# Autodesk Inventor assembly: Top Crossbrace
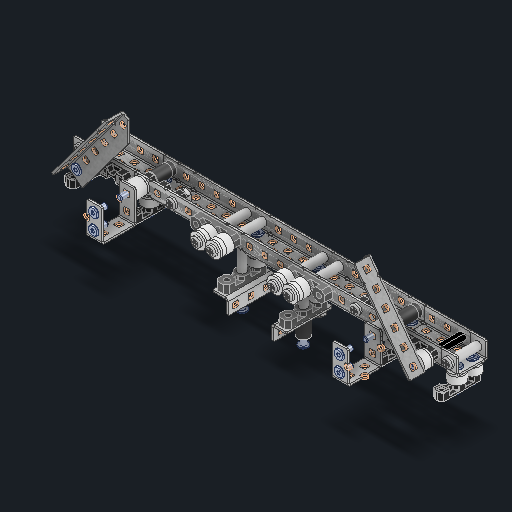
[picture p0: Inventor's stored thumbnail of the model, 512x512]
Saved by Autodesk Inventor 2025.1 (Build 291241000, 241)
## iProperties
Created: 2024-10-20
Part Number: Top Crossbrace
Document SubType Name: Assembly
Designer: Averey Ku
Author: Averey Ku
## Documents named in this file (41)
- C:\Users\avere\VEX\High Stakes\CAD\V3\Chassis\Structure\Top Crossbrace.iam
- C:\Users\avere\VEX\High Stakes\CAD\ROBOPROS-CAD-Inventor\Structure\C Channel\Aluminum 1x2x1\Alu C 1x2x1x17.ipt
- C:\Users\avere\VEX\High Stakes\CAD\ROBOPROS-CAD-Inventor\Structure\C Channel\Aluminum 2x2x2\Alu C 2x2x2x1.ipt
- C:\Users\avere\VEX\High Stakes\CAD\ROBOPROS-CAD-Inventor\Motion\Spacers\Spacer Nylon .500 OD\NSpacer White .500 OD x .375.ipt
- C:\Users\avere\VEX\High Stakes\CAD\ROBOPROS-CAD-Inventor\Motion\Shaft LS\Bearing Flat Low Profile.ipt
- C:\Users\avere\VEX\High Stakes\CAD\ROBOPROS-CAD-Inventor\Motion\Spacers\Washer Steel\SWasher .500 OD x .062500\SWasher .500 OD x .062500.ipt
- C:\Users\avere\VEX\High Stakes\CAD\ROBOPROS-CAD-Inventor\Motion\Spacers\Spacer Nylon .375 OD\NSpacer .375 OD x .125.ipt
- C:\Users\avere\VEX\High Stakes\CAD\ROBOPROS-CAD-Inventor\Motion\Spacers\Spacer Nylon .375 OD\NSpacer .375 OD x .500.ipt
- C:\Users\avere\VEX\High Stakes\CAD\ROBOPROS-CAD-Inventor\Structure\Hardware\Screw Steel - Star\SScrew Star Smooth 1.750.ipt
- C:\Users\avere\VEX\High Stakes\CAD\ROBOPROS-CAD-Inventor\Structure\Hardware\Screw Shoulder Robosource\SScrew Shoulder Smooth .375 x .12.ipt
- C:\Users\avere\VEX\High Stakes\CAD\ROBOPROS-CAD-Inventor\Motion\Spacers\Spacer Nylon .500 OD\NSpacer White .500 OD x .250.ipt
- C:\Users\avere\VEX\High Stakes\CAD\ROBOPROS-CAD-Inventor\Structure\Hardware\Screw Steel - Star\SScrew Star Smooth .750.ipt
- C:\Users\avere\VEX\High Stakes\CAD\ROBOPROS-CAD-Inventor\Structure\C Channel\Aluminum 1x2x1\Alu C 1x2x1x23.ipt
- C:\Users\avere\VEX\High Stakes\CAD\ROBOPROS-CAD-Inventor\Structure\Standoff\Standoff .875.ipt
- C:\Users\avere\VEX\High Stakes\CAD\ROBOPROS-CAD-Inventor\Structure\C Channel\Aluminum 1x3x1 Half Thick Cut\Alu C Half Thick 1x3x1x6.ipt
- C:\Users\avere\VEX\High Stakes\CAD\ROBOPROS-CAD-Inventor\Structure\Hardware\Screw Steel - Star\SScrew Star Smooth .875.ipt
- C:\Users\avere\VEX\High Stakes\CAD\ROBOPROS-CAD-Inventor\Structure\Hardware\Screw Steel - Star\SScrew Star Smooth .290.ipt
- C:\Users\avere\VEX\High Stakes\CAD\V3\Chassis\Structure\Right\Alu C 2x2x2x1 Right.ipt
- C:\Users\avere\VEX\High Stakes\CAD\V3\Chassis\Structure\Right\Bearing Flat Low Profile Right.ipt
- C:\Users\avere\VEX\High Stakes\CAD\V3\Chassis\Structure\Right\Alu C Half Thick 1x3x1x6 Right.ipt
- C:\Users\avere\VEX\High Stakes\CAD\ROBOPROS-CAD-Inventor\Motion\Spacers\Spacer Nylon .500 OD.ipt
- C:\Users\avere\VEX\High Stakes\CAD\ROBOPROS-CAD-Inventor\Motion\Spacers\Washer Steel\SWasher .500 OD x .062500.ipt
- C:\Users\avere\VEX\High Stakes\CAD\ROBOPROS-CAD-Inventor\Motion\Spacers\Spacer Nylon .375 OD.ipt
- C:\Users\avere\VEX\High Stakes\CAD\ROBOPROS-CAD-Inventor\Structure\Hardware\Screw Steel - Star.ipt
- C:\Users\avere\VEX\High Stakes\CAD\ROBOPROS-CAD-Inventor\Structure\Hardware\Screw Shoulder Robosource.ipt
- C:\Users\avere\VEX\High Stakes\CAD\ROBOPROS-CAD-Inventor\Structure\Standoff.ipt
- C:\Users\avere\VEX\High Stakes\CAD\ROBOPROS-CAD-Inventor\Motion\Spacers\Spacer Nylon .500 OD\NSpacer White .500 OD x .500.ipt
- C:\Users\avere\VEX\High Stakes\CAD\ROBOPROS-CAD-Inventor\Structure\Angle\Aluminum 1x1\Alu Angle 1x1x3.ipt
- C:\Users\avere\VEX\High Stakes\CAD\ROBOPROS-CAD-Inventor\Motion\Shaft LS\Bearing Flat.ipt
- C:\Users\avere\VEX\High Stakes\CAD\ROBOPROS-CAD-Inventor\Structure\C Channel\Aluminum 1x2x1\Alu C 1x2x1x25.ipt
- C:\Users\avere\VEX\High Stakes\CAD\ROBOPROS-CAD-Inventor\Structure\Nylon Standoff Rounded\Nylon Standoff .750.ipt
- C:\Users\avere\VEX\High Stakes\CAD\ROBOPROS-CAD-Inventor\Structure\Hardware\Screw Steel - Star\SScrew Star Smooth .250.ipt
- C:\Users\avere\VEX\High Stakes\CAD\ROBOPROS-CAD-Inventor\Structure\Hardware\Screw Steel - Star\SScrew Star Smooth 1.250.ipt
- C:\Users\avere\VEX\High Stakes\CAD\ROBOPROS-CAD-Inventor\Structure\Hardware\Nut Nylon Thread-Forming.ipt
- C:\Users\avere\VEX\High Stakes\CAD\ROBOPROS-CAD-Inventor\Structure\Hardware\Screw Steel - Star\SScrew Star Smooth 1.500.ipt
- C:\Users\avere\VEX\High Stakes\CAD\ROBOPROS-CAD-Inventor\Structure\Nylon Standoff Rounded\Nylon Standoff .875.ipt
- C:\Users\avere\VEX\High Stakes\CAD\ROBOPROS-CAD-Inventor\Structure\Hardware\Screw Nylon - Pan Head\NScrew Pan Head Threaded .250.ipt
- C:\Users\avere\VEX\High Stakes\CAD\ROBOPROS-CAD-Inventor\Structure\Hardware\Screw Nylon - Pan Head\NScrew Pan Head Threaded 1.000.ipt
- C:\Users\avere\VEX\High Stakes\CAD\ROBOPROS-CAD-Inventor\Structure\Hardware\Screw Nylon - Pan Head\NScrew Pan Head Threaded .500.ipt
- C:\Users\avere\VEX\High Stakes\CAD\ROBOPROS-CAD-Inventor\Structure\Hardware\Nut Nylon\Nut Nylon - White.ipt
- C:\Users\avere\VEX\High Stakes\CAD\ROBOPROS-CAD-Inventor\Structure\Hardware\Nut Nylon.ipt
## Components (119 placed, 33 different names)
1. Alu C 1x2x1x23:1 — Insert:23, Flush:2, Insert:33, Insert:34, Mate:6, Insert:39, Insert:40, Insert:79, Mate:12, Insert:80, Mate:13, Mate:14
2. Alu C 1x2x1x17:1 — Insert:3, Insert:5, Mate:2, Insert:15, Flush:1, Flush:2
3. NSpacer White .500 OD x .500:24 — Mate:10, Insert:116, Insert:123
4. Alu Angle 1x1x3:1 — Mate:9, Insert:115, Mate:16, Insert:119, Insert:129
5. NSpacer White .500 OD x .500:28 — Mate:9, Insert:114, Insert:124
6. Alu Angle 1x1x3:2 — Mate:10, Insert:118, Mate:17, Insert:120, Insert:130
7. Bearing Flat:1 — Insert:77, Insert:78, Insert:80, Mate:13
8. Bearing Flat:2 — Insert:75, Insert:76, Insert:79
9. NSpacer White .500 OD x .250:29 — Insert:76, Insert:88
10. NSpacer White .500 OD x .250:30 — Insert:75, Mate:12, Insert:85
11. NSpacer White .500 OD x .250:31 — Insert:78, Insert:92
12. NSpacer White .500 OD x .250:32 — Insert:77, Insert:90
13. NSpacer White .500 OD x .375:33 — Insert:85, Insert:86
14. SWasher .500 OD x .062500:6 — Insert:86, Insert:150
15. NSpacer White .500 OD x .375:35 — Insert:88
16. SWasher .500 OD x .062500:7 — Insert:149
17. NSpacer White .500 OD x .375:36 — Insert:90
18. SWasher .500 OD x .062500:8 — Insert:148
19. NSpacer White .500 OD x .375:37 — Insert:92
20. SWasher .500 OD x .062500:9 — Insert:147
21. Alu C 1x2x1x25:1 — Insert:97, Mate:14, Insert:98, Insert:99, Insert:100, Insert:101, Insert:102, Insert:103, Insert:104, Mate:15, Insert:114, Insert:116, Insert:121, Insert:122, Insert:125, Insert:126, Insert:127, Insert:128, Insert:133, Insert:134, Insert:135, Insert:136, Insert:137, Insert:138, Insert:139, Insert:140, Insert:141, Insert:142, Insert:143, Insert:144, Insert:145, Insert:146, Insert:152, Insert:153
22. SWasher .500 OD x .062500:10 — Insert:106
23. SWasher .500 OD x .062500:11 — Insert:105
24. SWasher .500 OD x .062500:12 — Insert:107
25. SWasher .500 OD x .062500:13 — Insert:108
26. SWasher .500 OD x .062500:14 — Insert:110
27. SWasher .500 OD x .062500:15 — Insert:109
28. SWasher .500 OD x .062500:16 — Insert:111
29. SWasher .500 OD x .062500:17 — Insert:112
30. Bearing Flat:4 — Insert:115, Mate:16
31. Bearing Flat:5 — Insert:118, Mate:17
32. NSpacer .375 OD x .500:5 — Insert:120, Insert:132
33. NSpacer .375 OD x .500:6 — Insert:119, Insert:131
34. Nylon Standoff .750:1 — Insert:121
35. Nylon Standoff .750:2 — Insert:122
36. NSpacer White .500 OD x .250:42 — Insert:124
37. NSpacer White .500 OD x .250:43 — Insert:123
38. SScrew Star Smooth .250:31 — Insert:125
39. SScrew Star Smooth .250:32 — Insert:126
40. SScrew Star Smooth 1.250:33 — Insert:127
41. SScrew Star Smooth 1.250:34 — Insert:128
42. Nut Nylon Thread-Forming:1 — Insert:130
43. Nut Nylon Thread-Forming:2 — Insert:129
44. SScrew Star Smooth 1.500:35 — Insert:131
45. SScrew Star Smooth 1.500:36 — Insert:132
46. Nylon Standoff .875:1 — Insert:133
47. Nylon Standoff .875:2 — Insert:134
48. Nylon Standoff .875:3 — Insert:135
49. Nylon Standoff .875:4 — Insert:136
50. NScrew Pan Head Threaded .250:1 — Insert:138
51. NScrew Pan Head Threaded .250:2 — Insert:139
52. NScrew Pan Head Threaded .250:3 — Insert:137
53. NScrew Pan Head Threaded .250:4 — Insert:140
54. Nylon Standoff .875:5 — Insert:141
55. NScrew Pan Head Threaded .250:5 — Insert:142
56. NScrew Pan Head Threaded .250:6 — Insert:143
57. Nylon Standoff .875:6 — Insert:146
58. NScrew Pan Head Threaded .250:7 — Insert:144
59. NScrew Pan Head Threaded .250:8 — Insert:145
60. NScrew Pan Head Threaded 1.000:1 — Insert:147
61. NScrew Pan Head Threaded 1.000:2 — Insert:148
62. NScrew Pan Head Threaded 1.000:3 — Insert:149
63. NScrew Pan Head Threaded 1.000:4 — Insert:150
64. NScrew Pan Head Threaded .500:1 — Insert:152
65. Nut Nylon - White:1 — Insert:151
66. NScrew Pan Head Threaded .500:2 — Insert:153
67. Nut Nylon - White:2 — Insert:154
68. SScrew Shoulder Smooth .375 x .12:3 — Insert:52
69. Alu C 2x2x2x1:1 — Insert:2, Insert:16, Insert:52
70. NSpacer White .500 OD x .375:1 — Insert:2, Insert:4
71. Bearing Flat Low Profile:1 — Insert:3, Mate:2, Insert:12, Insert:151
72. SWasher .500 OD x .062500:1 — Insert:4, Insert:5, Insert:23
73. NSpacer .375 OD x .125:1 — Insert:11
74. NSpacer .375 OD x .500:2 — Insert:11, Insert:12
75. SScrew Star Smooth 1.750:1 — Insert:15
76. SScrew Shoulder Smooth .375 x .12:1 — Insert:16
77. Alu C Half Thick 1x3x1x6:1 — Insert:33, Insert:36, Insert:38
78. Bearing Flat Low Profile:8 — Insert:34, Mate:6, Insert:37
79. NSpacer White .500 OD x .250:14 — Insert:36
80. SWasher .500 OD x .062500:3 — Insert:37
81. SScrew Star Smooth .875:14 — Insert:38
82. Standoff .875:1 — Insert:39
83. SScrew Star Smooth .290:15 — Insert:40, Insert:97
84. SScrew Shoulder Smooth .375 x .12:4 — Insert:53
85. Alu C 2x2x2x1 Right:1 — Insert:41, Insert:45, Insert:53
86. NSpacer White .500 OD x .375:15 — Insert:41, Insert:42
87. Bearing Flat Low Profile Right:1 — Insert:43, Insert:154
88. SWasher .500 OD x .062500:4 — Insert:42
89. NSpacer .375 OD x .125:3 — Insert:44
90. NSpacer .375 OD x .500:4 — Insert:43, Insert:44
91. SScrew Star Smooth 1.750:16
92. SScrew Shoulder Smooth .375 x .12:2 — Insert:45
93. Alu C Half Thick 1x3x1x6 Right:1 — Insert:48, Insert:50
94. Bearing Flat Low Profile Right:3 — Insert:49
95. NSpacer White .500 OD x .250:18 — Insert:48
96. SWasher .500 OD x .062500:5 — Insert:49
97. SScrew Star Smooth .875:19 — Insert:50
98. Standoff .875:2
99. SScrew Star Smooth .290:20
100. NSpacer White .500 OD x .250:6 — Insert:31, Insert:99, Insert:109
101. SScrew Star Smooth .750:6 — Insert:101
102. Bearing Flat Low Profile:4 — Insert:31
103. NSpacer White .500 OD x .250:7 — Insert:98, Insert:110
104. SScrew Star Smooth .750:7 — Insert:100
105. NSpacer White .500 OD x .250:38 — Insert:112
106. SScrew Star Smooth .750:27
107. Bearing Flat Low Profile:9
108. NSpacer White .500 OD x .250:39 — Insert:111
109. SScrew Star Smooth .750:28
110. NSpacer White .500 OD x .250:16 — Insert:47, Mate:15, Insert:106
111. SScrew Star Smooth .750:17 — Insert:102
112. Bearing Flat Low Profile Right:2 — Insert:46, Insert:47
113. SScrew Star Smooth .750:18 — Insert:103
114. NSpacer White .500 OD x .250:17 — Insert:46, Insert:104, Insert:105
115. NSpacer White .500 OD x .250:40 — Insert:107
116. SScrew Star Smooth .750:29
117. Bearing Flat Low Profile Right:4
118. SScrew Star Smooth .750:30
119. NSpacer White .500 OD x .250:41 — Insert:108
## Component patterns: (2 elements, first: NSpacer White .500 OD x .250:6 + SScrew Star Smooth .750:6 + Bearing Flat Low Profile:4 + NSpacer White .500 OD x .250:7 + SScrew Star Smooth .750:7), (2 elements, first: NSpacer White .500 OD x .250:16 + SScrew Star Smooth .750:17 + Bearing Flat Low Profile Right:2 + SScrew Star Smooth .750:18 + NSpacer White .500 OD x .250:17)
## Relationships (114: Insert 100, Mate 12, Flush 2)
- [Mate]: Alu C 1x2x1x17:1 ↔ Alu C 2x2x2x1:1
- Insert:2: Alu C 2x2x2x1:1 ↔ NSpacer White .500 OD x .375:1
- Insert:3: Alu C 1x2x1x17:1 ↔ Bearing Flat Low Profile:1
- Insert:4: NSpacer White .500 OD x .375:1 ↔ SWasher .500 OD x .062500:1
- Insert:5: Alu C 1x2x1x17:1 ↔ SWasher .500 OD x .062500:1
- Mate:2: Alu C 1x2x1x17:1 ↔ Bearing Flat Low Profile:1
- Insert:11: NSpacer .375 OD x .125:1 ↔ NSpacer .375 OD x .500:2
- Insert:12 (1.27 mm): Bearing Flat Low Profile:1 ↔ NSpacer .375 OD x .500:2
- Insert:15: Alu C 1x2x1x17:1 ↔ SScrew Star Smooth 1.750:1
- Insert:16: Alu C 2x2x2x1:1 ↔ SScrew Shoulder Smooth .375 x .12:1
- Flush:1 (-107.95 mm): Alu C 1x2x1x17:1
- Insert:23: Alu C 1x2x1x23:1 ↔ SWasher .500 OD x .062500:1
- Flush:2: Alu C 1x2x1x23:1 ↔ Alu C 1x2x1x17:1
- [Mate]: NSpacer White .500 OD x .250:6 ↔ Bearing Flat Low Profile:4
- [Insert] (1.27 mm): Bearing Flat Low Profile:4 ↔ NSpacer White .500 OD x .250:7
- Insert:31 (1.27 mm): NSpacer White .500 OD x .250:6 ↔ Bearing Flat Low Profile:4
- Insert:33 (14.2875 mm): Alu C 1x2x1x23:1 ↔ Alu C Half Thick 1x3x1x6:1
- Insert:34: Alu C 1x2x1x23:1 ↔ Bearing Flat Low Profile:8
- Mate:6: Alu C 1x2x1x23:1 ↔ Bearing Flat Low Profile:8
- Insert:36: Alu C Half Thick 1x3x1x6:1 ↔ NSpacer White .500 OD x .250:14
- Insert:37 (1.27 mm): Bearing Flat Low Profile:8 ↔ SWasher .500 OD x .062500:3
- Insert:38: Alu C Half Thick 1x3x1x6:1 ↔ SScrew Star Smooth .875:14
- Insert:39: Alu C 1x2x1x23:1 ↔ Standoff .875:1
- Insert:40: Alu C 1x2x1x23:1 ↔ SScrew Star Smooth .290:15
- Insert:41: Alu C 2x2x2x1 Right:1 ↔ NSpacer White .500 OD x .375:15
- Insert:42: NSpacer White .500 OD x .375:15 ↔ SWasher .500 OD x .062500:4
- Insert:43 (1.27 mm): Bearing Flat Low Profile Right:1 ↔ NSpacer .375 OD x .500:4
- Insert:44: NSpacer .375 OD x .125:3 ↔ NSpacer .375 OD x .500:4
- Insert:45: Alu C 2x2x2x1 Right:1 ↔ SScrew Shoulder Smooth .375 x .12:2
- Insert:46 (1.27 mm): Bearing Flat Low Profile Right:2 ↔ NSpacer White .500 OD x .250:17
- Insert:47 (1.27 mm): NSpacer White .500 OD x .250:16 ↔ Bearing Flat Low Profile Right:2
- Insert:48: Alu C Half Thick 1x3x1x6 Right:1 ↔ NSpacer White .500 OD x .250:18
- Insert:49 (1.27 mm): Bearing Flat Low Profile Right:3 ↔ SWasher .500 OD x .062500:5
- Insert:50: Alu C Half Thick 1x3x1x6 Right:1 ↔ SScrew Star Smooth .875:19
- Insert:52: SScrew Shoulder Smooth .375 x .12:3 ↔ Alu C 2x2x2x1:1
- Insert:53: SScrew Shoulder Smooth .375 x .12:4 ↔ Alu C 2x2x2x1 Right:1
- Mate:9: Alu Angle 1x1x3:1 ↔ NSpacer White .500 OD x .500:28
- Mate:10: NSpacer White .500 OD x .500:24 ↔ Alu Angle 1x1x3:2
- Insert:75: Bearing Flat:2 ↔ NSpacer White .500 OD x .250:30
- Insert:76: Bearing Flat:2 ↔ NSpacer White .500 OD x .250:29
- Insert:77: Bearing Flat:1 ↔ NSpacer White .500 OD x .250:32
- Insert:78: Bearing Flat:1 ↔ NSpacer White .500 OD x .250:31
- Insert:79: Alu C 1x2x1x23:1 ↔ Bearing Flat:2
- Mate:12: Alu C 1x2x1x23:1 ↔ NSpacer White .500 OD x .250:30
- Insert:80: Alu C 1x2x1x23:1 ↔ Bearing Flat:1
- Mate:13: Alu C 1x2x1x23:1 ↔ Bearing Flat:1
- Insert:85: NSpacer White .500 OD x .250:30 ↔ NSpacer White .500 OD x .375:33
- Insert:86: NSpacer White .500 OD x .375:33 ↔ SWasher .500 OD x .062500:6
- [Insert]: NSpacer White .500 OD x .375:35 ↔ SWasher .500 OD x .062500:7
- Insert:88: NSpacer White .500 OD x .250:29 ↔ NSpacer White .500 OD x .375:35
- [Insert]: NSpacer White .500 OD x .375:36 ↔ SWasher .500 OD x .062500:8
- Insert:90: NSpacer White .500 OD x .250:32 ↔ NSpacer White .500 OD x .375:36
- [Insert]: NSpacer White .500 OD x .375:37 ↔ SWasher .500 OD x .062500:9
- Insert:92: NSpacer White .500 OD x .250:31 ↔ NSpacer White .500 OD x .375:37
- Insert:97: Alu C 1x2x1x25:1 ↔ SScrew Star Smooth .290:15
- Mate:14: Alu C 1x2x1x23:1 ↔ Alu C 1x2x1x25:1
- Insert:98 (1.5875 mm): Alu C 1x2x1x25:1 ↔ NSpacer White .500 OD x .250:7
- Insert:99 (1.5875 mm): Alu C 1x2x1x25:1 ↔ NSpacer White .500 OD x .250:6
- Insert:100: Alu C 1x2x1x25:1 ↔ SScrew Star Smooth .750:7
- Insert:101: Alu C 1x2x1x25:1 ↔ SScrew Star Smooth .750:6
- Insert:102: Alu C 1x2x1x25:1 ↔ SScrew Star Smooth .750:17
- Insert:103: Alu C 1x2x1x25:1 ↔ SScrew Star Smooth .750:18
- Insert:104 (1.5875 mm): Alu C 1x2x1x25:1 ↔ NSpacer White .500 OD x .250:17
- Mate:15: Alu C 1x2x1x25:1 ↔ NSpacer White .500 OD x .250:16
- Insert:105: SWasher .500 OD x .062500:11 ↔ NSpacer White .500 OD x .250:17
- Insert:106: SWasher .500 OD x .062500:10 ↔ NSpacer White .500 OD x .250:16
- Insert:107: SWasher .500 OD x .062500:12 ↔ NSpacer White .500 OD x .250:40
- Insert:108: SWasher .500 OD x .062500:13 ↔ NSpacer White .500 OD x .250:41
- Insert:109: SWasher .500 OD x .062500:15 ↔ NSpacer White .500 OD x .250:6
- Insert:110: SWasher .500 OD x .062500:14 ↔ NSpacer White .500 OD x .250:7
- Insert:111: SWasher .500 OD x .062500:16 ↔ NSpacer White .500 OD x .250:39
- Insert:112: SWasher .500 OD x .062500:17 ↔ NSpacer White .500 OD x .250:38
- Insert:114: NSpacer White .500 OD x .500:28 ↔ Alu C 1x2x1x25:1
- Insert:115: Alu Angle 1x1x3:1 ↔ Bearing Flat:4
- Mate:16: Alu Angle 1x1x3:1 ↔ Bearing Flat:4
- Insert:116: NSpacer White .500 OD x .500:24 ↔ Alu C 1x2x1x25:1
- Insert:118: Alu Angle 1x1x3:2 ↔ Bearing Flat:5
- Mate:17: Alu Angle 1x1x3:2 ↔ Bearing Flat:5
- Insert:119: Alu Angle 1x1x3:1 ↔ NSpacer .375 OD x .500:6
- Insert:120: Alu Angle 1x1x3:2 ↔ NSpacer .375 OD x .500:5
- Insert:121: Alu C 1x2x1x25:1 ↔ Nylon Standoff .750:1
- Insert:122: Alu C 1x2x1x25:1 ↔ Nylon Standoff .750:2
- Insert:123: NSpacer White .500 OD x .500:24 ↔ NSpacer White .500 OD x .250:43
- Insert:124: NSpacer White .500 OD x .500:28 ↔ NSpacer White .500 OD x .250:42
- Insert:125: Alu C 1x2x1x25:1 ↔ SScrew Star Smooth .250:31
- Insert:126: Alu C 1x2x1x25:1 ↔ SScrew Star Smooth .250:32
- Insert:127: Alu C 1x2x1x25:1 ↔ SScrew Star Smooth 1.250:33
- Insert:128: Alu C 1x2x1x25:1 ↔ SScrew Star Smooth 1.250:34
- Insert:129: Alu Angle 1x1x3:1 ↔ Nut Nylon Thread-Forming:2
- Insert:130: Alu Angle 1x1x3:2 ↔ Nut Nylon Thread-Forming:1
- Insert:131 (6.35 mm): NSpacer .375 OD x .500:6 ↔ SScrew Star Smooth 1.500:35
- Insert:132 (6.35 mm): NSpacer .375 OD x .500:5 ↔ SScrew Star Smooth 1.500:36
- Insert:133: Alu C 1x2x1x25:1 ↔ Nylon Standoff .875:1
- Insert:134: Alu C 1x2x1x25:1 ↔ Nylon Standoff .875:2
- Insert:135: Alu C 1x2x1x25:1 ↔ Nylon Standoff .875:3
- Insert:136: Alu C 1x2x1x25:1 ↔ Nylon Standoff .875:4
- Insert:137: Alu C 1x2x1x25:1 ↔ NScrew Pan Head Threaded .250:3
- Insert:138: Alu C 1x2x1x25:1 ↔ NScrew Pan Head Threaded .250:1
- Insert:139: Alu C 1x2x1x25:1 ↔ NScrew Pan Head Threaded .250:2
- Insert:140: Alu C 1x2x1x25:1 ↔ NScrew Pan Head Threaded .250:4
- Insert:141: Alu C 1x2x1x25:1 ↔ Nylon Standoff .875:5
- Insert:142: Alu C 1x2x1x25:1 ↔ NScrew Pan Head Threaded .250:5
- Insert:143: Alu C 1x2x1x25:1 ↔ NScrew Pan Head Threaded .250:6
- Insert:144: Alu C 1x2x1x25:1 ↔ NScrew Pan Head Threaded .250:7
- Insert:145: Alu C 1x2x1x25:1 ↔ NScrew Pan Head Threaded .250:8
- Insert:146: Alu C 1x2x1x25:1 ↔ Nylon Standoff .875:6
- Insert:147: SWasher .500 OD x .062500:9 ↔ NScrew Pan Head Threaded 1.000:1
- Insert:148: SWasher .500 OD x .062500:8 ↔ NScrew Pan Head Threaded 1.000:2
- Insert:149: SWasher .500 OD x .062500:7 ↔ NScrew Pan Head Threaded 1.000:3
- Insert:150: SWasher .500 OD x .062500:6 ↔ NScrew Pan Head Threaded 1.000:4
- Insert:151 (1.27 mm): Nut Nylon - White:1 ↔ Bearing Flat Low Profile:1
- Insert:152: Alu C 1x2x1x25:1 ↔ NScrew Pan Head Threaded .500:1
- Insert:153: Alu C 1x2x1x25:1 ↔ NScrew Pan Head Threaded .500:2
- Insert:154 (1.27 mm): Nut Nylon - White:2 ↔ Bearing Flat Low Profile Right:1
## Named parameters: d46_d43 = 1.27 mm, d47_d31 = 0 mm, d134_d133 = 0 mm, d136_d134_d133 = 0 mm, d138_d136_d134_d133 = 0 mm
